# Autodesk Inventor assembly: EnsambleCajaElectrica
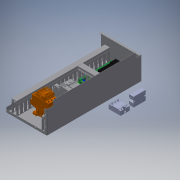
[picture p0: Inventor's stored thumbnail of the model, 180x180]
Saved by Autodesk Inventor 2017 (Build 210142000, 142)
## iProperties
Created: 2020-11-13
Part Number: EnsambleCajaElectrica
Document SubType Name: Assembly
Designer: USUARIO
Author: USUARIO
## Documents named in this file (10)
- D:\Laboratorio\Autoclave\Autoclave Horizontal\Sin Precamara\2019\Autoclave 40L con Vacio Angelica Castañeda #004588041 OP2019149\Modelo 3D\EnsambleCajaElectrica.iam
- D:\Laboratorio\Autoclave\Autoclave Horizontal\Sin Precamara\2019\Autoclave 40L con Vacio Angelica Castañeda #004588041 OP2019149\Modelo 3D\NextionControlV3.iam
- C:\Users\USUARIO\Documents\Inventor\Canaleta 30x60 450mm.iam
- C:\Users\USUARIO\Documents\Inventor\Canaleta 30x60 120mm.iam
- C:\Modelos 3D y DXF\Ex9C 25-38-NOARK.stp\Ex9C 25-38-NOARK.ipt
- C:\Modelos 3D y DXF\B1A-NOARK.stp\75856.ipt
- C:\Modelos 3D y DXF\Rele Relpol 2C\PZ8.ipt
- C:\Modelos 3D y DXF\B1A-NOARK.stp\B1A-NOARK.ipt
- C:\Modelos 3D y DXF\SSR\a24125pg.ipt
- D:\Laboratorio\Autoclave\Autoclave Horizontal\Sin Precamara\2019\Autoclave 40L con Vacio Angelica Castañeda #004588041 OP2019149\Modelo 3D\CAJA CONEXIONES ACH-40L-2019 MOD2020.ipt
## Components (11 placed, 9 different names)
1. NextionControlV3:1 [sub-assembly] — Mate:30, Mate:31
2. Canaleta 30x60 450mm:1 [sub-assembly] — Mate:9, Mate:14, Mate:18, Mate:20, Mate:22, Mate:23, Mate:25
3. Canaleta 30x60 120mm:1 [sub-assembly] — Mate:9, Mate:12, Mate:28
4. Canaleta 30x60 450mm:2 [sub-assembly] — Mate:12, Mate:26, Mate:27
5. Ex9C 25-38-NOARK:1 — Mate:14, Mate:29
6. 75856:1 — Mate:18
7. PZ8:1 — Mate:20
8. B1A-NOARK:1 — Mate:22
9. a24125pg:1
10. a24125pg:2
11. CAJA CONEXIONES ACH-40L-2019 MOD2020:1 — Mate:23, Mate:25, Mate:26, Mate:27, Mate:28, Mate:29, Mate:30, Mate:31
## Relationships (14: Mate 14)
- Mate:9: Canaleta 30x60 450mm:1 ↔ Canaleta 30x60 120mm:1
- Mate:12: Canaleta 30x60 120mm:1 ↔ Canaleta 30x60 450mm:2
- Mate:14 (95 mm): Canaleta 30x60 450mm:1 ↔ Ex9C 25-38-NOARK:1
- Mate:18 (22 mm): Canaleta 30x60 450mm:1 ↔ 75856:1
- Mate:20 (28 mm): Canaleta 30x60 450mm:1 ↔ PZ8:1
- Mate:22 (10 mm): Canaleta 30x60 450mm:1 ↔ B1A-NOARK:1
- Mate:23: Canaleta 30x60 450mm:1 ↔ CAJA CONEXIONES ACH-40L-2019 MOD2020:1
- Mate:25: Canaleta 30x60 450mm:1 ↔ CAJA CONEXIONES ACH-40L-2019 MOD2020:1
- Mate:26: Canaleta 30x60 450mm:2 ↔ CAJA CONEXIONES ACH-40L-2019 MOD2020:1
- Mate:27: Canaleta 30x60 450mm:2 ↔ CAJA CONEXIONES ACH-40L-2019 MOD2020:1
- Mate:28: Canaleta 30x60 120mm:1 ↔ CAJA CONEXIONES ACH-40L-2019 MOD2020:1
- Mate:29 (-2 mm): Ex9C 25-38-NOARK:1 ↔ CAJA CONEXIONES ACH-40L-2019 MOD2020:1
- Mate:30 (15 mm): NextionControlV3:1 ↔ CAJA CONEXIONES ACH-40L-2019 MOD2020:1
- Mate:31 (10 mm): NextionControlV3:1 ↔ CAJA CONEXIONES ACH-40L-2019 MOD2020:1
